# Autodesk Inventor assembly: Print_Parts_Fan_Holder
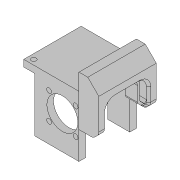
[picture p0: Inventor's stored thumbnail of the model, 180x180]
Saved by Autodesk Inventor 2020.1 (Build 241239000, 239)
## iProperties
Created: 2020-11-09
Part Number: Print_Parts_Fan_Holder
Document SubType Name: Assembly
Designer: kenta iguchi
Author: kenta iguchi
## Documents named in this file (3)
- D:\ken113\Documents\GitHub\Cheap_Belt_Printer\Model\Parts\Print_Parts\Rev2_Parts\Print_Parts_Fan_Holder.iam
- D:\ken113\Documents\GitHub\Cheap_Belt_Printer\Model\Parts\Print_Parts\Rev2_Parts\Print_Parts_H1.ipt
- D:\ken113\Documents\GitHub\Cheap_Belt_Printer\Model\Parts\Print_Parts\Rev2_Parts\Print_Parts_H2.ipt
## Components (2 placed, 2 different names)
1. Print_Parts_H1:1
2. Print_Parts_H2:1
## Relationships (2: Mate 1, Flush 1)
- [Mate]: Print_Parts_H1:1 ↔ Print_Parts_H2:1
- [Flush]: Print_Parts_H1:1 ↔ Print_Parts_H2:1
